# Autodesk Inventor assembly: Weapon (Motor-Side Pulley)
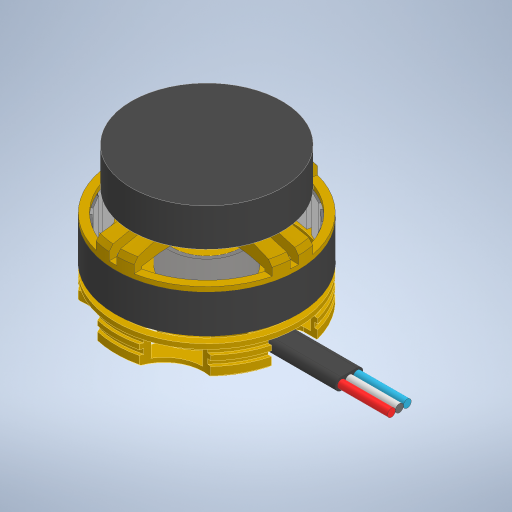
[picture p0: Inventor's stored thumbnail of the model, 512x512]
Saved by Autodesk Inventor 2023.2 (Build 272271000, 271)
## iProperties
Created: 2022-05-21
Part Number: Weapon (Motor-Side Pulley)
Document SubType Name: Assembly
Designer: Nathan Cai
Mass: 100 g
Surface Area: 105.713 cm^2
Volume: 11.2621 cm^3
Density: 8.87931 g/cm^3
Author: Nathan Cai
## Documents named in this file (3)
- C:\Users\Nathan Cai\Documents\Inventor\0.3rd Lawette - V3.6\Horizontal Weapon Assembly (Type U)\Weapon (Motor-Side Pulley).iam
- C:\Users\Nathan Cai\Documents\Inventor\0.3rd Lawette - V3.6\Horizontal Weapon Assembly (Type U)\Placeholder (Gear - M).ipt
- C:\Users\Nathan Cai\Documents\Inventor\0.3rd Lawette - V3.6\FEICHAO BE4108 380KV\FEICHAO BE4108 380KV.iam
## Components (2 placed, 2 different names)
1. Placeholder (Gear - M):1 — Mate:1, Mate:2
2. FEICHAO BE4108 380KV:1 [sub-assembly] — Mate:1, Mate:2
## Relationships (2: Mate 2)
- Mate:1: Placeholder (Gear - M):1 ↔ FEICHAO BE4108 380KV:1
- Mate:2 (-34.925 mm): Placeholder (Gear - M):1 ↔ FEICHAO BE4108 380KV:1
